# Autodesk Inventor assembly: ASY GBK 2120 short wall shield 2
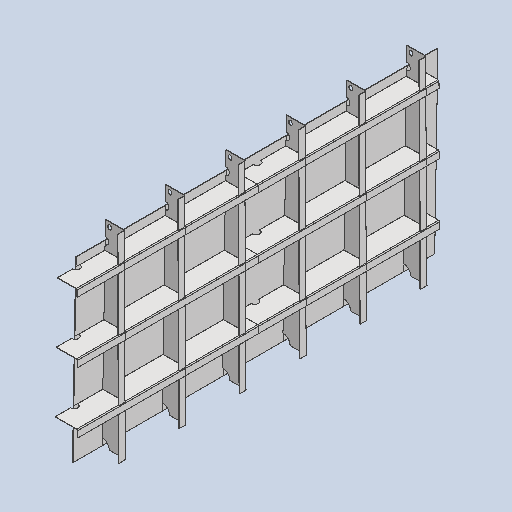
[picture p0: Inventor's stored thumbnail of the model, 512x512]
Saved by Autodesk Inventor 2026 (Build 300175000, 175)
## iProperties
Created: 2026-05-07
Part Number: ASY GBK 2120 short wall shield 2
Document SubType Name: Assembly
Designer: pokla
Stock Number: 1112
Mass: 272186 g
Surface Area: 175796 cm^2
Volume: 34673.3 cm^3
Density: 7.85 g/cm^3
Author: admin
## Documents named in this file (6)
- C:\Users\pokla\Documents\Inventor\GBK-Gubkinskiy\ASY GBK 2120 short wall shield 2.iam
- C:\Users\pokla\Documents\Inventor\GBK-Gubkinskiy\GBK 0101 main rib.ipt
- C:\Users\pokla\Documents\Inventor\GBK-Gubkinskiy\GBK 0102 stringer 1.ipt
- C:\Users\pokla\Documents\Inventor\GBK-Gubkinskiy\GBK 0103 stringer 2.ipt
- C:\Users\pokla\Documents\Inventor\GBK-Gubkinskiy\GBK 0104 stringer 3.ipt
- C:\Users\pokla\Documents\Inventor\GBK-Gubkinskiy\GBK 2121 shield 2.ipt
## Components (13 placed, 5 different names)
1. GBK 0102 stringer 1.ipt:1 — Жесткий:1, Жесткий:4
2. GBK 0102 stringer 1.ipt:2 — Жесткий:1
3. GBK 0103 stringer 2.ipt:1 — Жесткий:2, Жесткий:5
4. GBK 0103 stringer 2.ipt:2 — Жесткий:2
5. GBK 0104 stringer 3.ipt:1 — Жесткий:3, Жесткий:6
6. GBK 0104 stringer 3.ipt:2 — Жесткий:3
7. GBK 2121 shield 2.ipt:1 — Совмещение:2, Совмещение:1, Заподлицо:1
8. GBK 0101 main rib.ipt:1 — Совмещение:2, Совмещение:1, Заподлицо:1, Жесткий:6, Жесткий:5, Жесткий:4
9. GBK 0101 main rib.ipt:2
10. GBK 0101 main rib.ipt:3
11. GBK 0101 main rib.ipt:4
12. GBK 0101 main rib.ipt:5
13. GBK 0101 main rib.ipt:6
## Component patterns: (6 elements, first: GBK 0101 main rib.ipt:1)
## Relationships (9: WeldJoint 6, Mate 2, Flush 1)
- Совмещение:2 [Mate]: GBK 2121 shield 2.ipt:1 ↔ GBK 0101 main rib.ipt:1
- Совмещение:1 [Mate]: GBK 2121 shield 2.ipt:1 ↔ GBK 0101 main rib.ipt:1
- Заподлицо:1 [Flush] (254 mm): GBK 2121 shield 2.ipt:1 ↔ GBK 0101 main rib.ipt:1
- Жесткий:1 [WeldJoint]: GBK 0102 stringer 1.ipt:1 ↔ GBK 0102 stringer 1.ipt:2
- Жесткий:2 [WeldJoint]: GBK 0103 stringer 2.ipt:1 ↔ GBK 0103 stringer 2.ipt:2
- Жесткий:3 [WeldJoint]: GBK 0104 stringer 3.ipt:1 ↔ GBK 0104 stringer 3.ipt:2
- Жесткий:6 [WeldJoint] (4 mm): GBK 0104 stringer 3.ipt:1 ↔ GBK 0101 main rib.ipt:1
- Жесткий:5 [WeldJoint] (4 mm): GBK 0103 stringer 2.ipt:1 ↔ GBK 0101 main rib.ipt:1
- Жесткий:4 [WeldJoint] (4 mm): GBK 0102 stringer 1.ipt:1 ↔ GBK 0101 main rib.ipt:1
## Named parameters: основание_длина_нижнего = 196 mm, основание_длина_верхнего = 96 mm, стрингер_глубина_1 = 186.70056 mm, стрингер_глубина_2 = 175.35977 mm, стрингер_глубина_3 = 164.01899 mm, стрингер_глубина_4 = 152.6782 mm, стрингер_глубина_5 = 141.33742 mm, стрингер_глубина_6 = 129.99663 mm, стрингер_глубина_7 = 118.65585 mm, стрингер_глубина_8 = 107.31507 mm, Лист_ширина = 1480 mm, ребро_усилителей = 60 mm, паз_под_стрингер_глубина = 70 mm, паз_под_стрингер_толщина = 5 mm, отступ_от_пола_до_первого_стрингера = 410 mm, шаг_стрингеров = 500 mm, радиус_выреза_под_сварку = 30 mm, нахлест_шпангоутов_1_2 = 150 mm, нахлест_шпангоутов_2_3 = 120 mm, Стрингер_длина = 1490 mm, Лист_длина = 2980 mm, Шаг_шпангоутов = 496.66667 mm
